# Autodesk Inventor assembly: 2AM-17-A-0200 - slider motor and gearbox
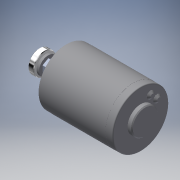
[picture p0: Inventor's stored thumbnail of the model, 180x180]
Saved by Autodesk Inventor 2017 (Build 210142000, 142)
## iProperties
Created: 2017-12-28
Part Number: 2AM-17-A-0200 - slider motor and gearbox
Document SubType Name: Assembly
Designer: Micah
Author: Micah
## Documents named in this file (6)
- C:\Users\Micah\Desktop\inventor\CADathon-2017\2AM-17-A-0200 - Smokestack Elevator\2AM-17-A-7200 - slider motor and gearbox.iam
- C:\Users\Micah\Desktop\inventor\COTS\Motors\Mini CIM Motor\217-3371-STEP.ipt
- C:\Users\Micah\Desktop\inventor\CADathon-2017\2AM-17-A-0200 - Smokestack Elevator\COTS\217-2761-STEP.ipt
- C:\Users\Micah\Desktop\inventor\CADathon-2017\2AM-17-A-0200 - Smokestack Elevator\COTS\217-3255-STEP.ipt
- C:\Users\Micah\Desktop\inventor\CADathon-2017\2AM-17-A-0200 - Smokestack Elevator\COTS\217-2737.20121205.ipt
- C:\Users\Micah\Desktop\inventor\CADathon-2017\2AM-17-A-0200 - Smokestack Elevator\2AM-17-P-7201 - sproket thing ig.ipt
## Components (6 placed, 5 different names)
1. 217-3371-STEP:1 — Mate:1, Insert:1, Rotational:2, Rotational:3, Rotational:4
2. 217-2761-STEP:2 — Mate:1
3. 217-3255-STEP:1 — Insert:1
4. 217-2737.20121205:1 — Rotational:2
5. 217-2737.20121205:2 — Rotational:3
6. 2AM-17-P-7201 - sproket thing ig:1 — Rotational:4
## Relationships (5: RevoluteJoint 3, Mate 1, Insert 1)
- Mate:1: 217-3371-STEP:1 ↔ 217-2761-STEP:2
- Insert:1 (-28.575 mm): 217-3371-STEP:1 ↔ 217-3255-STEP:1
- Rotational:2 [RevoluteJoint] (-11.43 mm): 217-3371-STEP:1 ↔ 217-2737.20121205:1
- Rotational:3 [RevoluteJoint] (-24.13 mm): 217-3371-STEP:1 ↔ 217-2737.20121205:2
- Rotational:4 [RevoluteJoint] (-15.24 mm): 217-3371-STEP:1 ↔ 2AM-17-P-7201 - sproket thing ig:1
